# Autodesk Inventor assembly: Flexipod2.0_2021_1_3
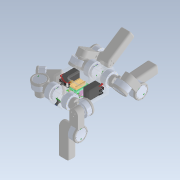
[picture p0: Inventor's stored thumbnail of the model, 180x180]
Saved by Autodesk Inventor 2020 (Build 240168000, 168)
## iProperties
Created: 2021-01-03
Part Number: Flexipod2.0_2021_1_3
Document SubType Name: Assembly
Designer: DELL
Author: DELL
## Documents named in this file (12)
- F:\SoftRobot2.0\FlexipodHardware2.0\FlexipodHardware\Flexipod2.0\robot_2021_1_3\Flexipod2.0_2021_1_3.iam
- F:\SoftRobot2.0\FlexipodHardware2.0\FlexipodHardware\Flexipod2.0\RMD_X6_stator.ipt
- F:\SoftRobot2.0\FlexipodHardware2.0\FlexipodHardware\Flexipod2.0\RMD_X6_rotor.ipt
- F:\SoftRobot2.0\FlexipodHardware2.0\FlexipodHardware\Flexipod2.0\robot_2021_1_3\thigh_link.ipt
- F:\SoftRobot2.0\FlexipodHardware2.0\FlexipodHardware\Flexipod2.0\robot_2021_1_3\shank_link.ipt
- F:\SoftRobot2.0\FlexipodHardware2.0\FlexipodHardware\Flexipod2.0\robot_2021_1_3\hip_link_4.ipt
- F:\SoftRobot2.0\FlexipodHardware2.0\FlexipodHardware\Flexipod2.0\robot_2021_1_3\hip_link_4_mirror.ipt
- F:\SoftRobot2.0\FlexipodHardware2.0\FlexipodHardware\Flexipod2.0\robot_2021_1_3\thigh_link_mirror.ipt
- F:\SoftRobot2.0\FlexipodHardware2.0\FlexipodHardware\Flexipod2.0\Jetson nano v2- Inventor\Jetson_Nano_Dev_Kit_3D_b01.iam
- F:\SoftRobot2.0\FlexipodHardware2.0\FlexipodHardware\Flexipod2.0\battery_6s_1550_ovonic.ipt
- F:\SoftRobot2.0\FlexipodHardware2.0\FlexipodHardware\Flexipod2.0\robot_2021_1_3\body.ipt
- F:\SoftRobot2.0\FlexipodHardware2.0\FlexipodHardware\Flexipod2.0\Arducam Camera.ipt
## Components (42 placed, 11 different names)
1. RMD_X6_stator:1 — Mate:1, Flush:1, Mate:19, Mate:85, Mate:86, Mate:87
2. RMD_X6_rotor:1 — Mate:1, Flush:1, Mate:20, Mate:21
3. RMD_X6_stator:2 — Mate:13, Mate:14, Mate:15, Mate:16
4. RMD_X6_rotor:2 — Mate:17, Mate:18
5. RMD_X6_stator:3 — Mate:10, Mate:22, Mate:23, Mate:24, Angle:3
6. RMD_X6_rotor:3 — Mate:11, Mate:12
7. thigh_link:1 — Mate:10, Mate:11, Mate:12, Mate:13, Mate:14, Mate:15, Angle:10
8. shank_link:1 — Mate:16, Mate:17, Mate:18
9. hip_link_4:1 — Mate:19, Mate:20, Mate:21, Mate:22, Mate:23, Mate:24
10. hip_link_4_mirror:1 — Mate:27, Mate:28, Mate:29, Mate:31, Mate:32, Mate:33
11. RMD_X6_stator:4 — Mate:27, Mate:82, Mate:83, Mate:84
12. RMD_X6_rotor:4 — Mate:28, Mate:29
13. RMD_X6_stator:5 — Mate:31, Mate:32, Mate:33, Mate:34, Angle:4
14. RMD_X6_rotor:5 — Mate:35, Mate:36
15. thigh_link_mirror:1 — Mate:34, Mate:35, Mate:36, Mate:41, Mate:42, Mate:43, Angle:8
16. RMD_X6_stator:6 — Mate:41, Mate:42, Mate:43
17. RMD_X6_rotor:6
18. shank_link:2
19. RMD_X6_stator:7 — Mate:91, Mate:92, Mate:93
20. RMD_X6_rotor:7
21. RMD_X6_stator:8
22. RMD_X6_rotor:8
23. RMD_X6_stator:9 — Angle:1
24. RMD_X6_rotor:9
25. thigh_link:2 — Angle:7
26. shank_link:3
27. hip_link_4:2
28. hip_link_4_mirror:2
29. RMD_X6_stator:10 — Mate:88, Mate:89, Mate:90
30. RMD_X6_rotor:10
31. RMD_X6_stator:11 — Angle:2
32. RMD_X6_rotor:11
33. thigh_link_mirror:2 — Angle:9
34. RMD_X6_stator:12
35. RMD_X6_rotor:12
36. shank_link:4
37. Jetson_Nano_Dev_Kit_3D_b01:1 [sub-assembly]
38. battery_6s_1550_ovonic:1
39. battery_6s_1550_ovonic:2
40. body:1 — Flush:13, Flush:14, Mate:81, Mate:82, Mate:83, Mate:84, Mate:85, Mate:86, Mate:87, Mate:88, Mate:89, Mate:90, Mate:91, Mate:92, Mate:93, Mate:94, Mate:95, Angle:5, Mate:96, Mate:97, Angle:6
41. Arducam Camera:1 — Mate:94, Mate:95, Angle:5
42. Arducam Camera:2 — Mate:96, Mate:97, Angle:6
## Relationships (113: Mate 89, Flush 14, Angle 10)
- Mate:1: RMD_X6_stator:1 ↔ RMD_X6_rotor:1
- Flush:1 (-3 mm): RMD_X6_stator:1 ↔ RMD_X6_rotor:1
- [Mate]: RMD_X6_stator:2 ↔ RMD_X6_rotor:2
- [Flush] (-3 mm): RMD_X6_stator:2 ↔ RMD_X6_rotor:2
- [Mate]: RMD_X6_stator:3 ↔ RMD_X6_rotor:3
- [Flush] (-3 mm): RMD_X6_stator:3 ↔ RMD_X6_rotor:3
- Mate:10: RMD_X6_stator:3 ↔ thigh_link:1
- Mate:11: RMD_X6_rotor:3 ↔ thigh_link:1
- Mate:12: RMD_X6_rotor:3 ↔ thigh_link:1
- Mate:13: RMD_X6_stator:2 ↔ thigh_link:1
- Mate:14: RMD_X6_stator:2 ↔ thigh_link:1
- Mate:15: RMD_X6_stator:2 ↔ thigh_link:1
- Mate:16: RMD_X6_stator:2 ↔ shank_link:1
- Mate:17: RMD_X6_rotor:2 ↔ shank_link:1
- Mate:18: RMD_X6_rotor:2 ↔ shank_link:1
- Mate:19: RMD_X6_stator:1 ↔ hip_link_4:1
- Mate:20: RMD_X6_rotor:1 ↔ hip_link_4:1
- Mate:21: RMD_X6_rotor:1 ↔ hip_link_4:1
- Mate:22: RMD_X6_stator:3 ↔ hip_link_4:1
- Mate:23: RMD_X6_stator:3 ↔ hip_link_4:1
- Mate:24: RMD_X6_stator:3 ↔ hip_link_4:1
- [Mate]: RMD_X6_stator:4 ↔ RMD_X6_rotor:4
- [Flush] (-3 mm): RMD_X6_stator:4 ↔ RMD_X6_rotor:4
- Mate:27: hip_link_4_mirror:1 ↔ RMD_X6_stator:4
- Mate:28: hip_link_4_mirror:1 ↔ RMD_X6_rotor:4
- Mate:29: hip_link_4_mirror:1 ↔ RMD_X6_rotor:4
- [Mate]: RMD_X6_stator:5 ↔ RMD_X6_rotor:5
- [Flush] (-3 mm): RMD_X6_stator:5 ↔ RMD_X6_rotor:5
- Mate:31: hip_link_4_mirror:1 ↔ RMD_X6_stator:5
- Mate:32: hip_link_4_mirror:1 ↔ RMD_X6_stator:5
- Mate:33: hip_link_4_mirror:1 ↔ RMD_X6_stator:5
- Mate:34: RMD_X6_stator:5 ↔ thigh_link_mirror:1
- Mate:35: RMD_X6_rotor:5 ↔ thigh_link_mirror:1
- Mate:36: RMD_X6_rotor:5 ↔ thigh_link_mirror:1
- [Mate]: RMD_X6_stator:6 ↔ RMD_X6_rotor:6
- [Flush] (-3 mm): RMD_X6_stator:6 ↔ RMD_X6_rotor:6
- [Mate]: RMD_X6_stator:6 ↔ shank_link:2
- [Mate]: RMD_X6_rotor:6 ↔ shank_link:2
- [Mate]: RMD_X6_rotor:6 ↔ shank_link:2
- Mate:41: thigh_link_mirror:1 ↔ RMD_X6_stator:6
- Mate:42: thigh_link_mirror:1 ↔ RMD_X6_stator:6
- Mate:43: thigh_link_mirror:1 ↔ RMD_X6_stator:6
- [Mate]: RMD_X6_stator:7 ↔ RMD_X6_rotor:7
- [Flush] (-3 mm): RMD_X6_stator:7 ↔ RMD_X6_rotor:7
- [Mate]: RMD_X6_stator:8 ↔ RMD_X6_rotor:8
- [Flush] (-3 mm): RMD_X6_stator:8 ↔ RMD_X6_rotor:8
- [Mate]: RMD_X6_stator:9 ↔ RMD_X6_rotor:9
- [Flush] (-3 mm): RMD_X6_stator:9 ↔ RMD_X6_rotor:9
- [Mate]: RMD_X6_stator:9 ↔ thigh_link:2
- [Mate]: RMD_X6_rotor:9 ↔ thigh_link:2
- [Mate]: RMD_X6_rotor:9 ↔ thigh_link:2
- [Mate]: RMD_X6_stator:8 ↔ thigh_link:2
- [Mate]: RMD_X6_stator:8 ↔ thigh_link:2
- [Mate]: RMD_X6_stator:8 ↔ thigh_link:2
- [Mate]: RMD_X6_stator:8 ↔ shank_link:3
- [Mate]: RMD_X6_rotor:8 ↔ shank_link:3
- [Mate]: RMD_X6_rotor:8 ↔ shank_link:3
- [Mate]: RMD_X6_stator:7 ↔ hip_link_4:2
- [Mate]: RMD_X6_rotor:7 ↔ hip_link_4:2
- [Mate]: RMD_X6_rotor:7 ↔ hip_link_4:2
- [Mate]: RMD_X6_stator:9 ↔ hip_link_4:2
- [Mate]: RMD_X6_stator:9 ↔ hip_link_4:2
- [Mate]: RMD_X6_stator:9 ↔ hip_link_4:2
- [Mate]: RMD_X6_stator:10 ↔ RMD_X6_rotor:10
- [Flush] (-3 mm): RMD_X6_stator:10 ↔ RMD_X6_rotor:10
- [Mate]: hip_link_4_mirror:2 ↔ RMD_X6_stator:10
- [Mate]: hip_link_4_mirror:2 ↔ RMD_X6_rotor:10
- [Mate]: hip_link_4_mirror:2 ↔ RMD_X6_rotor:10
- [Mate]: RMD_X6_stator:11 ↔ RMD_X6_rotor:11
- [Flush] (-3 mm): RMD_X6_stator:11 ↔ RMD_X6_rotor:11
- [Mate]: hip_link_4_mirror:2 ↔ RMD_X6_stator:11
- [Mate]: hip_link_4_mirror:2 ↔ RMD_X6_stator:11
- [Mate]: hip_link_4_mirror:2 ↔ RMD_X6_stator:11
- [Mate]: RMD_X6_stator:11 ↔ thigh_link_mirror:2
- [Mate]: RMD_X6_rotor:11 ↔ thigh_link_mirror:2
- [Mate]: RMD_X6_rotor:11 ↔ thigh_link_mirror:2
- [Mate]: RMD_X6_stator:12 ↔ RMD_X6_rotor:12
- [Flush] (-3 mm): RMD_X6_stator:12 ↔ RMD_X6_rotor:12
- [Mate]: RMD_X6_stator:12 ↔ shank_link:4
- [Mate]: RMD_X6_rotor:12 ↔ shank_link:4
- [Mate]: RMD_X6_rotor:12 ↔ shank_link:4
- [Mate]: thigh_link_mirror:2 ↔ RMD_X6_stator:12
- [Mate]: thigh_link_mirror:2 ↔ RMD_X6_stator:12
- [Mate]: thigh_link_mirror:2 ↔ RMD_X6_stator:12
- Angle:1 (30 deg): RMD_X6_stator:9
- Angle:2 (0 deg): RMD_X6_stator:11
- Angle:3 (180 deg): RMD_X6_stator:3
- Angle:4 (180 deg): RMD_X6_stator:5
- Flush:13: body:1
- Flush:14: body:1
- Mate:81: body:1
- Mate:82: RMD_X6_stator:4 ↔ body:1
- Mate:83: RMD_X6_stator:4 ↔ body:1
- Mate:84: RMD_X6_stator:4 ↔ body:1
- Mate:85: RMD_X6_stator:1 ↔ body:1
- Mate:86: RMD_X6_stator:1 ↔ body:1
- Mate:87: RMD_X6_stator:1 ↔ body:1
- Mate:88: RMD_X6_stator:10 ↔ body:1
- Mate:89: RMD_X6_stator:10 ↔ body:1
- Mate:90: RMD_X6_stator:10 ↔ body:1
- Mate:91: RMD_X6_stator:7 ↔ body:1
- Mate:92: RMD_X6_stator:7 ↔ body:1
- Mate:93: RMD_X6_stator:7 ↔ body:1
- Mate:94: body:1 ↔ Arducam Camera:1
- Mate:95: body:1 ↔ Arducam Camera:1
- Angle:5 (0 deg): body:1 ↔ Arducam Camera:1
- Mate:96: body:1 ↔ Arducam Camera:2
- Mate:97: body:1 ↔ Arducam Camera:2
- Angle:6 (0 deg): body:1 ↔ Arducam Camera:2
- Angle:7 (320 deg): thigh_link:2
- Angle:8 (0 deg): thigh_link_mirror:1
- Angle:9 (220 deg): thigh_link_mirror:2
- Angle:10 (180 deg): thigh_link:1
## Named parameters: d2_d0 = 0 mm, d3_d1 = -3 mm, d4_d0 = 0 mm, d5_d1 = -3 mm, d28_d0 = 0 mm, d29_d1 = -3 mm, d34_d4_d0 = 0 mm, d35_d5_d1 = -3 mm, d42_d2_d0 = 0 mm, d43_d3_d1 = -3 mm, d44_d19 = 0 mm, d45_d20 = 0 mm, d46_d21 = 0 mm, d50_d4_d0 = 0 mm, d51_d5_d1 = -3 mm, d52_d13 = 0 mm, d53_d14 = 0 mm, d54_d15 = 0 mm, d55_d16 = 0 mm, d56_d17 = 0 mm, d57_d18 = 0 mm, d58_d0 = 0 mm, d59_d1 = -3 mm, d60_d2_d0 = 0 mm, d61_d3_d1 = -3 mm, d62_d33 = 0 mm, d63_d34_d4_d0 = 0 mm, d64_d35_d5_d1 = -3 mm, d65_d36 = 0 mm, d66_d37 = 0 mm, d67_d38 = 0 mm, d68_d39 = 0 mm, d69_d40 = 0 mm, d70_d41 = 0 mm, d71_d42_d2_d0 = 0 mm, d72_d43_d3_d1 = -3 mm, d73_d44_d19 = 0 mm, d74_d45_d20 = 0 mm, d75_d46_d21 = 0 mm, d76_d47 = 0 mm, d77_d48 = 0 mm, d78_d49 = 0 mm, d79_d19 = 0 mm, d80_d20 = 0 mm, d81_d21 = 0 mm, d82_d22 = 0 mm, d83_d23 = 0 mm, d84_d24 = 0 mm, d85_d25 = 0 mm, d86_d26 = 0 mm, d87_d27 = 0 mm, d88_d28_d0 = 0 mm, d89_d29_d1 = -3 mm, d91_d31 = 0 mm, d92_d32 = 0 mm
